# Autodesk Inventor assembly: rollerbottom
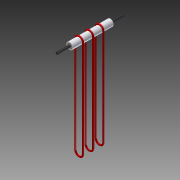
[picture p0: Inventor's stored thumbnail of the model, 180x180]
Saved by Autodesk Inventor 2011 SP1 (Build 150282100, 282)
## iProperties
Created: 2012-01-20
Part Number: rollerbottom
Document SubType Name: Assembly
Designer: Christopher
Author: Christopher
## Documents named in this file (5)
- C:\Users\Christopher\Documents\Christopher\FIRST\Inventor files\2012\tower bottom second design\rollerbottom.iam
- C:\Users\Christopher\Documents\Christopher\FIRST\Inventor files\2012\tower bottom second design\8 in pvc roller 1.379.ipt
- C:\Users\Christopher\Documents\Christopher\FIRST\Inventor files\2012\tower bottom second design\13 in axle.ipt
- C:\Users\Christopher\Documents\Christopher\FIRST\Inventor files\2012\tower bottom second design\axlebracetopvc.ipt
- C:\Users\Christopher\Documents\Christopher\FIRST\Inventor files\2012\tower bottom second design\17.5 in polycord 1.1.ipt
## Components (7 placed, 4 different names)
1. 8 in pvc roller 1.379:1 — Insert:1, Insert:2, Insert:4, Insert:5, Insert:6
2. 13 in axle:1 — Insert:3
3. axlebracetopvc:1 — Insert:1
4. axlebracetopvc:2 — Insert:2, Insert:3
5. 17.5 in polycord 1.1:1 — Insert:6, Flush:2
6. 17.5 in polycord 1.1:2 — Insert:5, Flush:1, Flush:2
7. 17.5 in polycord 1.1:3 — Insert:4, Flush:1
## Relationships (8: Insert 6, Flush 2)
- Insert:1: 8 in pvc roller 1.379:1 ↔ axlebracetopvc:1
- Insert:2: 8 in pvc roller 1.379:1 ↔ axlebracetopvc:2
- Insert:3 (63.5 mm): 13 in axle:1 ↔ axlebracetopvc:2
- Insert:4 (50.8 mm): 8 in pvc roller 1.379:1 ↔ 17.5 in polycord 1.1:3
- Insert:5 (101.6 mm): 8 in pvc roller 1.379:1 ↔ 17.5 in polycord 1.1:2
- Insert:6 (152.4 mm): 8 in pvc roller 1.379:1 ↔ 17.5 in polycord 1.1:1
- Flush:1: 17.5 in polycord 1.1:2 ↔ 17.5 in polycord 1.1:3
- Flush:2: 17.5 in polycord 1.1:1 ↔ 17.5 in polycord 1.1:2
